# Autodesk Inventor assembly: assymbly of steel and right side part
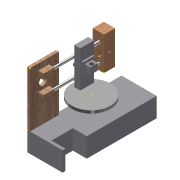
[picture p0: Inventor's stored thumbnail of the model, 180x180]
Saved by Autodesk Inventor 2019 (Build 230136000, 136)
## iProperties
Created: 2020-02-29
Part Number: assymbly of steel and right side part
Document SubType Name: Assembly
Designer: SHANKAR
Author: SHANKAR
## Documents named in this file (7)
- C:\Users\SHANKAR\Documents\assymbly of steel and right side part.iam
- C:\Users\SHANKAR\Documents\left side part.exploration.ipt
- C:\Users\SHANKAR\Documents\steel rod.exploration.ipt
- C:\Users\SHANKAR\Documents\right side part.ipt
- C:\Users\SHANKAR\Documents\final base part.ipt
- C:\Users\SHANKAR\Documents\tile rotation part.ipt
- C:\Users\SHANKAR\Documents\perfect rectangle.ipt
## Components (7 placed, 6 different names)
1. left side part.exploration:1 — Rigid:1, Rotational:1, Mate:1, Flush:1, Flush:2
2. steel rod.exploration:1 — Rigid:1, Cylindrical:1
3. steel rod.exploration:2 — Rotational:1
4. right side part:1 — Cylindrical:1
5. final base part:1 — Mate:1, Flush:1, Flush:2, Insert:1
6. tile rotation part:1 — Insert:1
7. perfect rectangle:1
## Relationships (7: Flush 2, WeldJoint 1, RevoluteJoint 1, CylindricalJoint 1, Mate 1, Insert 1)
- Rigid:1 [WeldJoint]: left side part.exploration:1 ↔ steel rod.exploration:1
- Rotational:1 [RevoluteJoint]: left side part.exploration:1 ↔ steel rod.exploration:2
- Cylindrical:1: steel rod.exploration:1 ↔ right side part:1
- Mate:1: left side part.exploration:1 ↔ final base part:1
- Flush:1: left side part.exploration:1 ↔ final base part:1
- Flush:2: left side part.exploration:1 ↔ final base part:1
- Insert:1: final base part:1 ↔ tile rotation part:1
